# Autodesk Inventor assembly: ASSEMBLY_Main
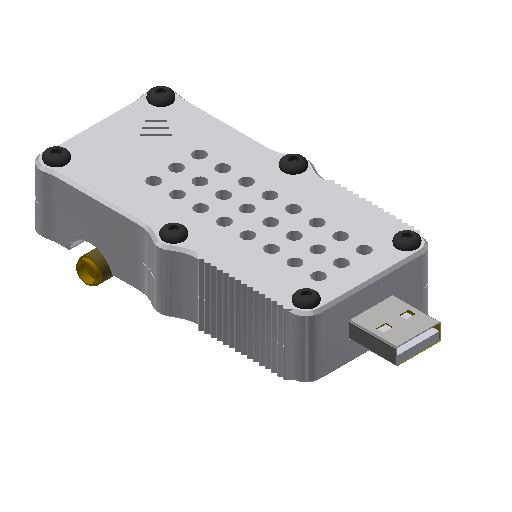
[picture p0: Inventor's stored thumbnail of the model, 512x512]
Saved by Autodesk Inventor 2025 (Build 290162010, 162A)
## iProperties
Created: 2018-09-08
Part Number: ASSEMBLY_Main
Document SubType Name: Assembly
Designer: Andrzej
Author: Andrzej
## Documents named in this file (5)
- D:\_ANDRZEJ_LACZEWSKI\_OTHER\MECH - RTL-SDR dongle case & some design tips for FDM technology\MCAD\1_REV1\ASSEMBLY_MAIN_REVA\ASSEMBLY_Main.iam
- D:\_ANDRZEJ_LACZEWSKI\_OTHER\MECH - RTL-SDR dongle case & some design tips for FDM technology\MCAD\1_REV1\ASSEMBLY_MAIN_REVA\3DP_PLA_Case_bottom_half.ipt
- D:\_ANDRZEJ_LACZEWSKI\_OTHER\MECH - RTL-SDR dongle case & some design tips for FDM technology\MCAD\1_REV1\__COTS_PARTS\COTS_GENERIC_rtl_sdr_dongle.ipt
- D:\_ANDRZEJ_LACZEWSKI\_OTHER\MECH - RTL-SDR dongle case & some design tips for FDM technology\MCAD\1_REV1\ASSEMBLY_MAIN_REVA\3DP_PLA_Case_top_half.ipt
- D:\_ANDRZEJ_LACZEWSKI\_OTHER\MECH - RTL-SDR dongle case & some design tips for FDM technology\MCAD\1_REV1\__COTS_PARTS\COTS_GENERIC_M3x16_screw.ipt
## Components (9 placed, 4 different names)
1. 3DP_PLA_Case_bottom_half:1 — Mate:1, Mate:2, Mate:3, Mate:4, Flush:1, Flush:2, Mate:17
2. COTS_GENERIC_rtl_sdr_dongle:1 — Mate:1, Mate:2, Mate:3
3. 3DP_PLA_Case_top_half:1 — Mate:4, Flush:1, Flush:2, Mate:5, Mate:6, Mate:7, Mate:8, Mate:9, Mate:10, Mate:11, Mate:12, Mate:13, Mate:14, Mate:15, Mate:16, Flush:3
4. COTS_GENERIC_M3x16_screw:1 — Mate:8, Mate:13
5. COTS_GENERIC_M3x16_screw:2 — Mate:6, Mate:11
6. COTS_GENERIC_M3x16_screw:3 — Mate:5, Mate:15
7. COTS_GENERIC_M3x16_screw:4 — Mate:10, Mate:16
8. COTS_GENERIC_M3x16_screw:5 — Mate:9, Mate:14
9. COTS_GENERIC_M3x16_screw:6 — Mate:7, Mate:12
## Relationships (20: Mate 17, Flush 3)
- Mate:1: 3DP_PLA_Case_bottom_half:1 ↔ COTS_GENERIC_rtl_sdr_dongle:1
- Mate:2 (0.25 mm): 3DP_PLA_Case_bottom_half:1 ↔ COTS_GENERIC_rtl_sdr_dongle:1
- Mate:3 (0.25 mm): 3DP_PLA_Case_bottom_half:1 ↔ COTS_GENERIC_rtl_sdr_dongle:1
- Mate:4: 3DP_PLA_Case_bottom_half:1 ↔ 3DP_PLA_Case_top_half:1
- Flush:1: 3DP_PLA_Case_bottom_half:1 ↔ 3DP_PLA_Case_top_half:1
- Flush:2: 3DP_PLA_Case_bottom_half:1 ↔ 3DP_PLA_Case_top_half:1
- Mate:5: 3DP_PLA_Case_top_half:1 ↔ COTS_GENERIC_M3x16_screw:3
- Mate:6: 3DP_PLA_Case_top_half:1 ↔ COTS_GENERIC_M3x16_screw:2
- Mate:7: 3DP_PLA_Case_top_half:1 ↔ COTS_GENERIC_M3x16_screw:6
- Mate:8: 3DP_PLA_Case_top_half:1 ↔ COTS_GENERIC_M3x16_screw:1
- Mate:9: 3DP_PLA_Case_top_half:1 ↔ COTS_GENERIC_M3x16_screw:5
- Mate:10: 3DP_PLA_Case_top_half:1 ↔ COTS_GENERIC_M3x16_screw:4
- Mate:11: 3DP_PLA_Case_top_half:1 ↔ COTS_GENERIC_M3x16_screw:2
- Mate:12: 3DP_PLA_Case_top_half:1 ↔ COTS_GENERIC_M3x16_screw:6
- Mate:13: 3DP_PLA_Case_top_half:1 ↔ COTS_GENERIC_M3x16_screw:1
- Mate:14: 3DP_PLA_Case_top_half:1 ↔ COTS_GENERIC_M3x16_screw:5
- Mate:15: 3DP_PLA_Case_top_half:1 ↔ COTS_GENERIC_M3x16_screw:3
- Mate:16: 3DP_PLA_Case_top_half:1 ↔ COTS_GENERIC_M3x16_screw:4
- Flush:3: 3DP_PLA_Case_top_half:1
- Mate:17: 3DP_PLA_Case_bottom_half:1
